# Autodesk Inventor assembly: capflipper
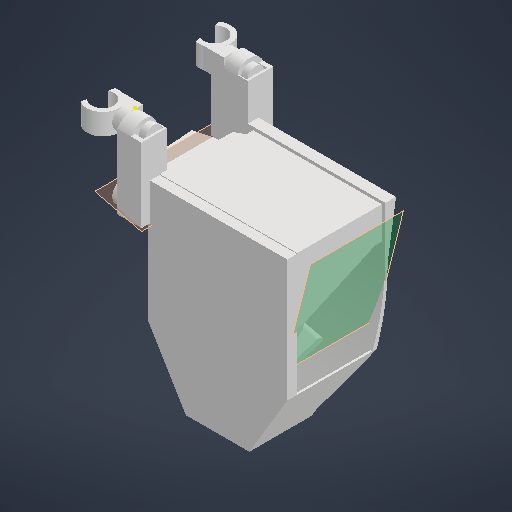
[picture p0: Inventor's stored thumbnail of the model, 512x512]
Saved by Autodesk Inventor 2026 (Build 300175050, 175E)
## iProperties
Created: 2026-05-08
Part Number: capflipper
Document SubType Name: Assembly
Designer: sniel
Author: sniel
## Documents named in this file (6)
- C:\Users\sniel\OneDrive\SDU\4_Semester\Applied automation\AppliedAutomationProject\feeder\capflipper.iam
- C:\Users\sniel\OneDrive\SDU\4_Semester\Applied automation\AppliedAutomationProject\feeder\capFlipperConnectionPoint.ipt
- C:\Users\sniel\OneDrive\SDU\4_Semester\Applied automation\AppliedAutomationProject\feeder\STEP\Wall v2\CapTurnerV1.ipt
- C:\Users\sniel\OneDrive\SDU\4_Semester\Applied automation\AppliedAutomationProject\feeder\Bottle.ipt
- C:\Users\sniel\OneDrive\SDU\4_Semester\Applied automation\AppliedAutomationProject\feeder\STEP\Wall v2\CapTurnerV2.ipt
- C:\Users\sniel\OneDrive\SDU\4_Semester\Applied automation\AppliedAutomationProject\feeder\STEP\Wall v2\Lid.ipt
## Components (6 placed, 5 different names)
1. capFlipperConnectionPoint:1 — Mate:1, Mate:2, Mate:3, Mate:5, Mate:6
2. CapTurnerV1:1 — Mate:1, Mate:2, Mate:3, Mate:4
3. Bottle:1 — Mate:4, Mate:7
4. CapTurnerV2:1 — Mate:5, Mate:6, Mate:7, Flush:1, Mate:8, Flush:2, Flush:3
5. Lid:1 — Flush:1, Flush:2, Flush:3
6. Bottle:2 — Mate:8
## Relationships (11: Mate 8, Flush 3)
- Mate:1: capFlipperConnectionPoint:1 ↔ CapTurnerV1:1
- Mate:2: capFlipperConnectionPoint:1 ↔ CapTurnerV1:1
- Mate:3 (0.25 mm): capFlipperConnectionPoint:1 ↔ CapTurnerV1:1
- Mate:4: CapTurnerV1:1 ↔ Bottle:1
- Mate:5: capFlipperConnectionPoint:1 ↔ CapTurnerV2:1
- Mate:6: capFlipperConnectionPoint:1 ↔ CapTurnerV2:1
- Mate:7: Bottle:1 ↔ CapTurnerV2:1
- Flush:1: CapTurnerV2:1 ↔ Lid:1
- Mate:8: CapTurnerV2:1 ↔ Bottle:2
- Flush:2: CapTurnerV2:1 ↔ Lid:1
- Flush:3: CapTurnerV2:1 ↔ Lid:1
